# Autodesk Inventor assembly: main pto gears
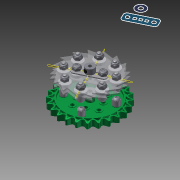
[picture p0: Inventor's stored thumbnail of the model, 180x180]
Saved by Autodesk Inventor 2014 SP1 (Build 180222100, 222)
## iProperties
Created: 2014-02-23
Part Number: main pto gears
Document SubType Name: Assembly
Designer: Ryan
Author: Ryan
## Documents named in this file (9)
- C:\Users\Ryan\Desktop\sw\toss up 4th robot\drive\main pto gears - ratchet.iam
- C:\Users\Ryan\Desktop\sw\lib\Aperture VEX CAD Library\Sprockets\green\High Strength 24-Tooth Sprocket.ipt
- C:\Users\Ryan\Desktop\sw\lib\Aperture VEX CAD Library\Hardware\8-32\8-32 nylock.ipt
- C:\Users\Ryan\Desktop\sw\lib\Aperture VEX CAD Library\Hardware\8-32\8-32_.500.ipt
- C:\Users\Ryan\Desktop\sw\lib\Aperture VEX CAD Library\Spacers\SPACER-0500-0250.ipt
- C:\Users\Ryan\Desktop\sw\lib\Aperture VEX CAD Library\Hardware\Shaft Collar.ipt
- C:\Users\Ryan\Desktop\sw\toss up 4th robot\drive\ratchet dog clutch.iam
- C:\Users\Ryan\Desktop\sw\lib\Aperture VEX CAD Library\Spacers\thin\SPACER-0320-0250.ipt
- C:\Users\Ryan\Desktop\sw\lib\Aperture VEX CAD Library\Spacers\SPACER-0500-0125.ipt
## Components (19 placed, 8 different names)
1. ratchet dog clutch:1 [sub-assembly] — Mate:14, Mate:25, Mate:26
2. High Strength 24-Tooth Sprocket:1 — Mate:5, Mate:7, Mate:8, Mate:9, Mate:10, Mate:17, Mate:23, Mate:24, Mate:25
3. SPACER-0500-0250:1 — Mate:9, Mate:10
4. Shaft Collar:2 — Mate:14
5. ratchet dog clutch:2 [sub-assembly] — Mate:17, Mate:18, Mate:19, Mate:27
6. Shaft Collar:3 — Mate:18, Mate:19
7. SPACER-0500-0125:2 — Mate:23, Mate:24, Mate:26, Mate:27
8. 8-32 nylock:1 — Mate:8
9. 8-32_.500:1
10. SPACER-0320-0250:1 — Mate:5, Mate:7
11. 8-32 nylock:2
12. 8-32_.500:2
13. SPACER-0320-0250:2
14. 8-32 nylock:3
15. 8-32_.500:3
16. SPACER-0320-0250:3
17. 8-32 nylock:4
18. 8-32_.500:4
19. SPACER-0320-0250:4
## Component patterns: (4 elements, first: 8-32 nylock:1 + 8-32_.500:1 + SPACER-0320-0250:1)
## Relationships (17: Mate 17)
- [Mate]: 8-32_.500:1 ↔ SPACER-0320-0250:1
- [Mate]: 8-32_.500:1 ↔ SPACER-0320-0250:1
- [Mate]: 8-32 nylock:1 ↔ 8-32_.500:1
- Mate:5: High Strength 24-Tooth Sprocket:1 ↔ SPACER-0320-0250:1
- Mate:7: High Strength 24-Tooth Sprocket:1 ↔ SPACER-0320-0250:1
- Mate:8: High Strength 24-Tooth Sprocket:1 ↔ 8-32 nylock:1
- Mate:9: High Strength 24-Tooth Sprocket:1 ↔ SPACER-0500-0250:1
- Mate:10: High Strength 24-Tooth Sprocket:1 ↔ SPACER-0500-0250:1
- Mate:14: ratchet dog clutch:1 ↔ Shaft Collar:2
- Mate:17: High Strength 24-Tooth Sprocket:1 ↔ ratchet dog clutch:2
- Mate:18: ratchet dog clutch:2 ↔ Shaft Collar:3
- Mate:19: ratchet dog clutch:2 ↔ Shaft Collar:3
- Mate:23: High Strength 24-Tooth Sprocket:1 ↔ SPACER-0500-0125:2
- Mate:24: High Strength 24-Tooth Sprocket:1 ↔ SPACER-0500-0125:2
- Mate:25: ratchet dog clutch:1 ↔ High Strength 24-Tooth Sprocket:1
- Mate:26: ratchet dog clutch:1 ↔ SPACER-0500-0125:2
- Mate:27 (12.7 mm): ratchet dog clutch:2 ↔ SPACER-0500-0125:2
